# Autodesk Inventor assembly: MagnetAssembly
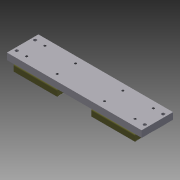
[picture p0: Inventor's stored thumbnail of the model, 180x180]
Saved by Autodesk Inventor 2012 (Build 160160000, 160)
## iProperties
Created: 2012-04-08
Part Number: MagnetAssembly
Document SubType Name: Assembly
Designer: admin
Mass: 387.861 g
Surface Area: 699.229 cm^2
Volume: 127.464 cm^3
Density: 3.04291 g/cm^3
Author: admin
## Documents named in this file (3)
- C:\Users\admin\Documents\Inventor\SumoJaime2012\MagnetAssembly.iam
- C:\Users\admin\Documents\Inventor\SumoJaime2012\TeflonMagnet.iam
- C:\Users\admin\Documents\Inventor\SumoJaime2012\MagnetPlate.ipt
## Components (5 placed, 2 different names)
1. TeflonMagnet:1 [sub-assembly] — Mate:4, Flush:4, Flush:5
2. TeflonMagnet:2 [sub-assembly] — Mate:3, Flush:2, Flush:3, Flush:7, Mate:5, Flush:8
3. TeflonMagnet:3 [sub-assembly] — Mate:4, Flush:4, Flush:5, Flush:6, Mate:6, Flush:9
4. TeflonMagnet:4 [sub-assembly] — Mate:3, Flush:2, Flush:3
5. MagnetPlate:1 — Flush:1, Mate:2, Flush:6, Flush:7, Mate:5, Mate:6, Flush:8, Flush:9
## Relationships (14: Flush 9, Mate 5)
- Flush:1: MagnetPlate:1
- Mate:2: MagnetPlate:1
- Mate:3 (7.62 mm): TeflonMagnet:2 ↔ TeflonMagnet:4
- Flush:2: TeflonMagnet:2 ↔ TeflonMagnet:4
- Flush:3: TeflonMagnet:2 ↔ TeflonMagnet:4
- Mate:4 (7.62 mm): TeflonMagnet:1 ↔ TeflonMagnet:3
- Flush:4: TeflonMagnet:1 ↔ TeflonMagnet:3
- Flush:5: TeflonMagnet:1 ↔ TeflonMagnet:3
- Flush:6: TeflonMagnet:3 ↔ MagnetPlate:1
- Flush:7: TeflonMagnet:2 ↔ MagnetPlate:1
- Mate:5: TeflonMagnet:2 ↔ MagnetPlate:1
- Mate:6: TeflonMagnet:3 ↔ MagnetPlate:1
- Flush:8 (9.525 mm): TeflonMagnet:2 ↔ MagnetPlate:1
- Flush:9 (9.525 mm): TeflonMagnet:3 ↔ MagnetPlate:1
